# Autodesk Inventor assembly: Test tube rack
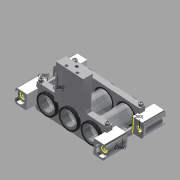
[picture p0: Inventor's stored thumbnail of the model, 180x180]
Saved by Autodesk Inventor 2017 (Build 210142000, 142)
## iProperties
Created: 2016-12-06
Part Number: Test tube rack
Document SubType Name: Assembly
Designer: qupec
Author: qupec
## Documents named in this file (11)
- C:\Users\qupec\Desktop\UMD Near Space\STAR\CAD\Mechanical\Test tube rack.iam
- C:\Users\qupec\Desktop\UMD Near Space\STAR\CAD\Mechanical\Tube Holder connector.ipt
- C:\Users\qupec\Desktop\UMD Near Space\STAR\CAD\Mechanical\Test Tube.ipt
- C:\Users\qupec\Desktop\UMD Near Space\STAR\CAD\Mechanical\Tube Holder with camera attachment.ipt
- C:\Users\qupec\Desktop\UMD Near Space\STAR\CAD\Mechanical\Tube grip.ipt
- C:\Users\qupec\Desktop\UMD Near Space\STAR\CAD\Mechanical\Tube Holder Halve.ipt
- C:\Users\qupec\Desktop\UMD Near Space\STAR\CAD\Mechanical\Tube Holder Halve 2.ipt
- C:\Users\qupec\Desktop\UMD Near Space\STAR\CAD\Mechanical\Tube Holder Halve 3.ipt
- C:\Users\qupec\Documents\Inventor\Content Center Files\R2017\en-US\U UNC 2603(1)\Unbrako - 4 x 1 - 48 - 1 - Unbrako.ipt
- C:\Users\qupec\Desktop\UMD Near Space\STAR\CAD\Mechanical\LINEAR SLEEVE BRNG.ipt
- C:\Users\qupec\Desktop\UMD Near Space\STAR\CAD\Mechanical\linear bearing.ipt
## Components (27 placed, 10 different names)
1. Tube Holder Halve:1 — Mate:10, Mate:11, Mate:21, Mate:23, Mate:46, Mate:53, Mate:57, Mate:59, Mate:61, Mate:64, Mate:65, Mate:68
2. Tube Holder Halve 2:1 — Mate:7, Mate:8, Mate:9, Mate:10, Mate:11, Mate:20, Mate:22, Mate:45, Mate:48, Mate:61, Mate:69, Mate:70, Mate:73
3. Tube grip:1 — Mate:3, Flush:6
4. Tube grip:2 — Mate:2, Flush:3
5. Tube grip:3 — Mate:4, Flush:5, Mate:8
6. Tube grip:4 — Mate:5, Flush:2, Mate:9
7. Tube grip:5 — Mate:1, Flush:4, Mate:7
8. Tube grip:6 — Mate:6, Flush:1
9. Test Tube:1 — Mate:5, Mate:6, Flush:1, Flush:2, Flush:13
10. Test Tube:2 — Mate:3, Mate:4, Flush:5, Flush:6, Flush:12
11. Test Tube:3 — Mate:1, Mate:2, Flush:3, Flush:4, Flush:11
12. Tube Holder connector:1 — Mate:20, Mate:22, Mate:36
13. Tube Holder connector:2 — Mate:21, Mate:23, Mate:24, Mate:25
14. Tube Holder with camera attachment:1 — Mate:24, Mate:25, Mate:26, Mate:27, Mate:55, Mate:56, Mate:58, Mate:60, Mate:62, Mate:63, Mate:66, Mate:67, Mate:71, Mate:72
15. Tube Holder Halve 3:1 — Mate:26, Mate:27, Mate:36, Flush:11, Flush:12, Flush:13, Mate:49, Mate:50, Mate:60
16. Unbrako UNC Hex Socket Cap - Inch 4 x 1 - Unbrako:1 — Mate:45, Mate:46, Mate:59
17. Unbrako UNC Hex Socket Cap - Inch 4 x 1 - Unbrako:2 — Mate:50, Mate:58
18. Unbrako UNC Hex Socket Cap - Inch 4 x 1 - Unbrako:3 — Mate:49, Mate:55, Mate:56
19. Unbrako UNC Hex Socket Cap - Inch 4 x 1 - Unbrako:4 — Mate:48, Mate:53, Mate:57
20. LINEAR SLEEVE BRNG:1 — Mate:74, Mate:79
21. LINEAR SLEEVE BRNG:2 — Mate:75, Mate:78
22. LINEAR SLEEVE BRNG:3 — Mate:77, Mate:80
23. LINEAR SLEEVE BRNG:4 — Mate:76, Mate:81
24. linear bearing:1 — Mate:62, Mate:66, Mate:72, Mate:76, Mate:81
25. linear bearing:2 — Mate:64, Mate:68, Mate:70, Mate:75, Mate:78
26. linear bearing:3 — Mate:63, Mate:67, Mate:71, Mate:74, Mate:79
27. linear bearing:4 — Mate:65, Mate:69, Mate:73, Mate:77, Mate:80
## Relationships (62: Mate 53, Flush 9)
- Mate:1: Tube grip:5 ↔ Test Tube:3
- Mate:2: Tube grip:2 ↔ Test Tube:3
- Mate:3: Tube grip:1 ↔ Test Tube:2
- Mate:4: Tube grip:3 ↔ Test Tube:2
- Mate:5: Tube grip:4 ↔ Test Tube:1
- Mate:6: Tube grip:6 ↔ Test Tube:1
- Flush:1: Tube grip:6 ↔ Test Tube:1
- Flush:2: Tube grip:4 ↔ Test Tube:1
- Flush:3: Tube grip:2 ↔ Test Tube:3
- Flush:4: Tube grip:5 ↔ Test Tube:3
- Flush:5: Tube grip:3 ↔ Test Tube:2
- Flush:6: Tube grip:1 ↔ Test Tube:2
- Mate:7: Tube Holder Halve 2:1 ↔ Tube grip:5
- Mate:8: Tube Holder Halve 2:1 ↔ Tube grip:3
- Mate:9: Tube Holder Halve 2:1 ↔ Tube grip:4
- Mate:10: Tube Holder Halve:1 ↔ Tube Holder Halve 2:1
- Mate:11: Tube Holder Halve:1 ↔ Tube Holder Halve 2:1
- Mate:20: Tube Holder Halve 2:1 ↔ Tube Holder connector:1
- Mate:21: Tube Holder Halve:1 ↔ Tube Holder connector:2
- Mate:22: Tube Holder Halve 2:1 ↔ Tube Holder connector:1
- Mate:23: Tube Holder Halve:1 ↔ Tube Holder connector:2
- Mate:24: Tube Holder connector:2 ↔ Tube Holder with camera attachment:1
- Mate:25: Tube Holder connector:2 ↔ Tube Holder with camera attachment:1
- Mate:26: Tube Holder with camera attachment:1 ↔ Tube Holder Halve 3:1
- Mate:27: Tube Holder with camera attachment:1 ↔ Tube Holder Halve 3:1
- Mate:36: Tube Holder connector:1 ↔ Tube Holder Halve 3:1
- Flush:11 (-3.175 mm): Test Tube:3 ↔ Tube Holder Halve 3:1
- Flush:12 (-3.175 mm): Test Tube:2 ↔ Tube Holder Halve 3:1
- Flush:13 (-3.175 mm): Test Tube:1 ↔ Tube Holder Halve 3:1
- Mate:45: Tube Holder Halve 2:1 ↔ Unbrako UNC Hex Socket Cap - Inch 4 x 1 - Unbrako:1
- Mate:46: Tube Holder Halve:1 ↔ Unbrako UNC Hex Socket Cap - Inch 4 x 1 - Unbrako:1
- Mate:48: Tube Holder Halve 2:1 ↔ Unbrako UNC Hex Socket Cap - Inch 4 x 1 - Unbrako:4
- Mate:49: Tube Holder Halve 3:1 ↔ Unbrako UNC Hex Socket Cap - Inch 4 x 1 - Unbrako:3
- Mate:50: Tube Holder Halve 3:1 ↔ Unbrako UNC Hex Socket Cap - Inch 4 x 1 - Unbrako:2
- Mate:53: Tube Holder Halve:1 ↔ Unbrako UNC Hex Socket Cap - Inch 4 x 1 - Unbrako:4
- Mate:55: Tube Holder with camera attachment:1 ↔ Unbrako UNC Hex Socket Cap - Inch 4 x 1 - Unbrako:3
- Mate:56: Tube Holder with camera attachment:1 ↔ Unbrako UNC Hex Socket Cap - Inch 4 x 1 - Unbrako:3
- Mate:57: Tube Holder Halve:1 ↔ Unbrako UNC Hex Socket Cap - Inch 4 x 1 - Unbrako:4
- Mate:58: Tube Holder with camera attachment:1 ↔ Unbrako UNC Hex Socket Cap - Inch 4 x 1 - Unbrako:2
- Mate:59: Tube Holder Halve:1 ↔ Unbrako UNC Hex Socket Cap - Inch 4 x 1 - Unbrako:1
- Mate:60: Tube Holder with camera attachment:1 ↔ Tube Holder Halve 3:1
- Mate:61: Tube Holder Halve:1 ↔ Tube Holder Halve 2:1
- Mate:62: Tube Holder with camera attachment:1 ↔ linear bearing:1
- Mate:63: Tube Holder with camera attachment:1 ↔ linear bearing:3
- Mate:64: Tube Holder Halve:1 ↔ linear bearing:2
- Mate:65: Tube Holder Halve:1 ↔ linear bearing:4
- Mate:66: Tube Holder with camera attachment:1 ↔ linear bearing:1
- Mate:67: Tube Holder with camera attachment:1 ↔ linear bearing:3
- Mate:68: Tube Holder Halve:1 ↔ linear bearing:2
- Mate:69: Tube Holder Halve 2:1 ↔ linear bearing:4
- Mate:70: Tube Holder Halve 2:1 ↔ linear bearing:2
- Mate:71: Tube Holder with camera attachment:1 ↔ linear bearing:3
- Mate:72: Tube Holder with camera attachment:1 ↔ linear bearing:1
- Mate:73: Tube Holder Halve 2:1 ↔ linear bearing:4
- Mate:74: LINEAR SLEEVE BRNG:1 ↔ linear bearing:3
- Mate:75: LINEAR SLEEVE BRNG:2 ↔ linear bearing:2
- Mate:76: LINEAR SLEEVE BRNG:4 ↔ linear bearing:1
- Mate:77: LINEAR SLEEVE BRNG:3 ↔ linear bearing:4
- Mate:78: LINEAR SLEEVE BRNG:2 ↔ linear bearing:2
- Mate:79: LINEAR SLEEVE BRNG:1 ↔ linear bearing:3
- Mate:80: LINEAR SLEEVE BRNG:3 ↔ linear bearing:4
- Mate:81: LINEAR SLEEVE BRNG:4 ↔ linear bearing:1
